# Autodesk Inventor assembly: Full Assembly
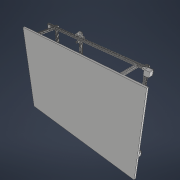
[picture p0: Inventor's stored thumbnail of the model, 180x180]
Saved by Autodesk Inventor 2022 (Build 260153000, 153)
## iProperties
Created: 2023-06-15
Part Number: Full Assembly
Document SubType Name: Assembly
Designer: Ryan Mitcham
Author: Ryan Mitcham
## Documents named in this file (21)
- C:\Users\Gaming\OneDrive\Documents\Inventor\XYZ-Gantry\Full Assembly.iam
- C:\Users\Gaming\OneDrive\Documents\Inventor\XYZ-Gantry\X-Axis.ipt
- C:\Users\Gaming\OneDrive\Documents\Inventor\XYZ-Gantry\XY-Axis Connection\XY-Axis Connection.iam
- C:\Users\Gaming\OneDrive\Documents\Inventor\XYZ-Gantry\Y-Axis.ipt
- C:\Users\Gaming\OneDrive\Documents\Inventor\XYZ-Gantry\YZ-Axis Connection\YZ-Axis Connection.iam
- C:\Users\Gaming\OneDrive\Documents\Inventor\XYZ-Gantry\Z-Axis.ipt
- C:\Users\Gaming\OneDrive\Documents\Inventor\XYZ-Gantry\Standard Parts\NEMA 17 Bi-Polar Stepper Motor.ipt
- C:\Users\Gaming\OneDrive\Documents\Inventor\XYZ-Gantry\Standard Parts\GT2 20 Teeth Motor Pulley.ipt
- C:\Users\Gaming\OneDrive\Documents\Inventor\XYZ-Gantry\Pulley Plates\X-Axis End - Straight.ipt
- C:\Users\Gaming\OneDrive\Documents\Inventor\XYZ-Gantry\Pulley Plates\Extrusion-compatible Spacer.ipt
- C:\Users\Gaming\OneDrive\Documents\Inventor\XYZ-Gantry\Standard Parts\GT2 20 Teeth Pulley.ipt
- C:\Users\Gaming\OneDrive\Documents\Inventor\XYZ-Gantry\Pulley Plates\X-Axis End - Corner.ipt
- C:\Users\Gaming\OneDrive\Documents\Inventor\XYZ-Gantry\Stepper Motor Mounting Plate.ipt
- C:\Users\Gaming\OneDrive\Documents\Inventor\XYZ-Gantry\Standard Parts\GT2 2-Side Belt Clamp.ipt
- C:\Users\Gaming\OneDrive\Documents\Inventor\XYZ-Gantry\Pulley Plates\Y-Axis Pulley Spacer.ipt
- C:\Users\Gaming\OneDrive\Documents\Inventor\XYZ-Gantry\Endstop Mounting Plate.ipt
- C:\Users\Gaming\OneDrive\Documents\Inventor\XYZ-Gantry\Support Structure\Horizontal Support.ipt
- C:\Users\Gaming\OneDrive\Documents\Inventor\XYZ-Gantry\Support Structure\Horizontal Support - Surround Bracket.ipt
- C:\Users\Gaming\OneDrive\Documents\Inventor\XYZ-Gantry\Main Carriage\Main Carriage.iam
- C:\Users\Gaming\OneDrive\Documents\Inventor\XYZ-Gantry\Support Structure\Vertical Support - with Brackets.iam
- C:\Users\Gaming\OneDrive\Documents\Inventor\XYZ-Gantry\Support Structure\Base Plate.ipt
## Components (58 placed, 20 different names)
1. X-Axis:1 — Flush:1, Flush:2, Mate:11, Mate:12, Mate:13, Mate:16, Mate:17, Flush:3, Mate:28, Flush:4, Mate:38, Flush:7, Flush:8, Flush:12, Mate:60, Mate:61, Mate:62, Mate:98, Flush:16, Mate:99, Mate:102, Flush:21, Flush:22, Mate:103, Flush:27, Mate:111, Mate:120, Flush:29, Mate:121, Flush:31
2. X-Axis:2 — Flush:1, Flush:2, Mate:14, Mate:15, Flush:5, Mate:33, Flush:6, Flush:9, Flush:10, Mate:43, Flush:11, Mate:52, Mate:53, Mate:54, Mate:79, Mate:106, Flush:23, Flush:24, Mate:108, Mate:110, Flush:26, Mate:118, Flush:28, Mate:123, Flush:32
3. XY-Axis Connection:1 [sub-assembly] — Mate:1, Mate:2, Mate:3, Mate:14, Mate:16, Mate:17
4. XY-Axis Connection:2 [sub-assembly] — Mate:4, Mate:5, Mate:6, Mate:7, Mate:15
5. Y-Axis:1 — Mate:1, Mate:2, Mate:3, Mate:4, Mate:5, Mate:6, Mate:7, Mate:18, Mate:19, Mate:77, Mate:78, Mate:96, Mate:97, Flush:18, Mate:100
6. YZ-Axis Connection:1 [sub-assembly] — Mate:18, Mate:19, Mate:22, Mate:23, Mate:24, Mate:48, Mate:49, Mate:50, Mate:73, Mate:74, Mate:75, Mate:76, Angle:1, Angle:2
7. NEMA 17 Bi-Polar Stepper Motor:1 — Mate:22, Mate:23, Mate:24, Mate:25, Mate:26
8. GT2 20 Teeth Motor Pulley:1 — Mate:25, Mate:26, Mate:51
9. X-Axis End - Straight:1 — Flush:3, Mate:28, Mate:29, Mate:30, Flush:4
10. Extrusion-compatible Spacer:1 — Mate:29, Mate:30, Mate:31, Mate:32
11. GT2 20 Teeth Pulley:1 — Mate:31, Mate:32
12. X-Axis End - Straight:2 — Flush:5, Mate:33, Flush:6, Mate:34, Mate:35
13. Extrusion-compatible Spacer:2 — Mate:34, Mate:35, Mate:36, Mate:37
14. GT2 20 Teeth Pulley:2 — Mate:36, Mate:37
15. X-Axis End - Corner:1 — Mate:38, Flush:7, Flush:8, Mate:39, Mate:40, Mate:104
16. Extrusion-compatible Spacer:3 — Mate:39, Mate:40, Mate:41, Mate:42
17. GT2 20 Teeth Pulley:3 — Mate:41, Mate:42
18. X-Axis End - Corner:2 — Flush:9, Flush:10, Mate:43, Mate:44, Mate:45, Mate:119
19. Extrusion-compatible Spacer:4 — Mate:44, Mate:45, Mate:46, Mate:47
20. GT2 20 Teeth Pulley:4 — Mate:46, Mate:47
21. Z-Axis:1 — Mate:48, Mate:49, Mate:50, Mate:51, Mate:68, Flush:13, Flush:14, Mate:101, Flush:19, Flush:20, Mate:114, Mate:115
22. Stepper Motor Mounting Plate:1 — Flush:11, Mate:52, Mate:53, Mate:54, Mate:55, Mate:56, Mate:57
23. NEMA 17 Bi-Polar Stepper Motor:2 — Mate:55, Mate:56, Mate:57, Mate:58, Mate:59
24. GT2 20 Teeth Motor Pulley:2 — Mate:58, Mate:59
25. Stepper Motor Mounting Plate:2 — Flush:12, Mate:60, Mate:61, Mate:62, Mate:63, Mate:64, Mate:65, Mate:122
26. NEMA 17 Bi-Polar Stepper Motor:3 — Mate:63, Mate:64, Mate:65, Mate:66, Mate:67
27. GT2 20 Teeth Motor Pulley:3 — Mate:66, Mate:67
28. X-Axis End - Straight:3 — Mate:68, Flush:13, Flush:14, Mate:69, Mate:70
29. Extrusion-compatible Spacer:5 — Mate:69, Mate:70, Mate:71, Mate:72
30. GT2 20 Teeth Pulley:5 — Mate:71, Mate:72
31. GT2 2-Side Belt Clamp:1 — Mate:73, Mate:74, Angle:2
32. GT2 2-Side Belt Clamp:2 — Mate:75, Mate:76, Angle:1
33. X-Axis End - Straight:4 — Mate:77, Mate:78, Mate:79, Mate:80, Mate:81, Mate:82, Mate:83
34. GT2 20 Teeth Pulley:6 — Mate:84, Mate:85
35. GT2 20 Teeth Pulley:7 — Mate:86, Mate:87
36. Y-Axis Pulley Spacer:1 — Mate:80, Mate:82, Mate:84, Mate:85
37. Y-Axis Pulley Spacer:2 — Mate:81, Mate:83, Mate:86, Mate:87
38. X-Axis End - Straight:5 — Mate:96, Mate:97, Mate:98, Flush:17
39. GT2 20 Teeth Pulley:8
40. GT2 20 Teeth Pulley:9
41. Y-Axis Pulley Spacer:3
42. Y-Axis Pulley Spacer:4
43. Endstop Mounting Plate:1 — Flush:16, Mate:99, Mate:113
44. Endstop Mounting Plate:2 — Flush:17, Flush:18, Mate:100
45. Endstop Mounting Plate:3 — Mate:101, Flush:19, Flush:20
46. Horizontal Support:1 — Mate:102, Flush:21, Mate:105, Mate:107
47. Horizontal Support - Surround Bracket:1 — Flush:22, Mate:103, Mate:104, Mate:105
48. Horizontal Support - Surround Bracket:2 — Mate:106, Flush:23, Mate:107
49. Horizontal Support:2 — Flush:24, Mate:108, Flush:25, Mate:109, Mate:112
50. Horizontal Support - Surround Bracket:3 — Flush:25, Mate:109, Mate:110, Flush:26
51. Horizontal Support - Surround Bracket:4 — Flush:27, Mate:111, Mate:112, Mate:113
52. Main Carriage:1 [sub-assembly] — Mate:114, Mate:115, Mate:116, Mate:117
53. GT2 2-Side Belt Clamp:3 — Mate:116, Mate:117
54. Vertical Support - with Brackets:1 [sub-assembly] — Mate:118, Flush:28, Mate:119, Flush:30
55. Vertical Support - with Brackets:2 [sub-assembly] — Mate:120, Flush:29, Flush:30
56. Vertical Support - with Brackets:3 [sub-assembly] — Mate:121, Flush:31, Mate:122, Flush:33
57. Vertical Support - with Brackets:4 [sub-assembly] — Mate:123, Flush:32, Flush:33, Mate:124, Flush:34, Flush:35
58. Base Plate:1 — Mate:124, Flush:34, Flush:35
## Relationships (154: Mate 118, Flush 34, Angle 2)
- Flush:1: X-Axis:1 ↔ X-Axis:2
- Flush:2: X-Axis:1 ↔ X-Axis:2
- Mate:1: XY-Axis Connection:1 ↔ Y-Axis:1
- Mate:2: XY-Axis Connection:1 ↔ Y-Axis:1
- Mate:3: XY-Axis Connection:1 ↔ Y-Axis:1
- Mate:4: XY-Axis Connection:2 ↔ Y-Axis:1
- Mate:5: XY-Axis Connection:2 ↔ Y-Axis:1
- Mate:6: XY-Axis Connection:2 ↔ Y-Axis:1
- Mate:7: XY-Axis Connection:2 ↔ Y-Axis:1
- Mate:11: X-Axis:1
- Mate:12: X-Axis:1
- Mate:13: X-Axis:1
- Mate:14 (1 mm): X-Axis:2 ↔ XY-Axis Connection:1
- Mate:15 (1 mm): X-Axis:2 ↔ XY-Axis Connection:2
- Mate:16 (1 mm): X-Axis:1 ↔ XY-Axis Connection:1
- Mate:17 (1 mm): X-Axis:1 ↔ XY-Axis Connection:1
- Mate:18 (1 mm): Y-Axis:1 ↔ YZ-Axis Connection:1
- Mate:19 (1 mm): Y-Axis:1 ↔ YZ-Axis Connection:1
- Mate:22: YZ-Axis Connection:1 ↔ NEMA 17 Bi-Polar Stepper Motor:1
- Mate:23: YZ-Axis Connection:1 ↔ NEMA 17 Bi-Polar Stepper Motor:1
- Mate:24: YZ-Axis Connection:1 ↔ NEMA 17 Bi-Polar Stepper Motor:1
- Mate:25 (10 mm): NEMA 17 Bi-Polar Stepper Motor:1 ↔ GT2 20 Teeth Motor Pulley:1
- Mate:26: NEMA 17 Bi-Polar Stepper Motor:1 ↔ GT2 20 Teeth Motor Pulley:1
- Flush:3: X-Axis:1 ↔ X-Axis End - Straight:1
- Mate:28: X-Axis:1 ↔ X-Axis End - Straight:1
- Mate:29: X-Axis End - Straight:1 ↔ Extrusion-compatible Spacer:1
- Mate:30: X-Axis End - Straight:1 ↔ Extrusion-compatible Spacer:1
- Mate:31: Extrusion-compatible Spacer:1 ↔ GT2 20 Teeth Pulley:1
- Mate:32: Extrusion-compatible Spacer:1 ↔ GT2 20 Teeth Pulley:1
- Flush:4 (20 mm): X-Axis:1 ↔ X-Axis End - Straight:1
- Flush:5: X-Axis:2 ↔ X-Axis End - Straight:2
- Mate:33: X-Axis:2 ↔ X-Axis End - Straight:2
- Flush:6 (-20 mm): X-Axis:2 ↔ X-Axis End - Straight:2
- Mate:34: X-Axis End - Straight:2 ↔ Extrusion-compatible Spacer:2
- Mate:35: X-Axis End - Straight:2 ↔ Extrusion-compatible Spacer:2
- Mate:36: Extrusion-compatible Spacer:2 ↔ GT2 20 Teeth Pulley:2
- Mate:37: Extrusion-compatible Spacer:2 ↔ GT2 20 Teeth Pulley:2
- Mate:38: X-Axis:1 ↔ X-Axis End - Corner:1
- Flush:7: X-Axis:1 ↔ X-Axis End - Corner:1
- Flush:8: X-Axis:1 ↔ X-Axis End - Corner:1
- Mate:39: X-Axis End - Corner:1 ↔ Extrusion-compatible Spacer:3
- Mate:40: X-Axis End - Corner:1 ↔ Extrusion-compatible Spacer:3
- Mate:41: Extrusion-compatible Spacer:3 ↔ GT2 20 Teeth Pulley:3
- Mate:42: Extrusion-compatible Spacer:3 ↔ GT2 20 Teeth Pulley:3
- Flush:9: X-Axis:2 ↔ X-Axis End - Corner:2
- Flush:10: X-Axis:2 ↔ X-Axis End - Corner:2
- Mate:43: X-Axis:2 ↔ X-Axis End - Corner:2
- Mate:44: X-Axis End - Corner:2 ↔ Extrusion-compatible Spacer:4
- Mate:45: X-Axis End - Corner:2 ↔ Extrusion-compatible Spacer:4
- Mate:46: Extrusion-compatible Spacer:4 ↔ GT2 20 Teeth Pulley:4
- Mate:47: Extrusion-compatible Spacer:4 ↔ GT2 20 Teeth Pulley:4
- Mate:48: YZ-Axis Connection:1 ↔ Z-Axis:1
- Mate:49 (-10 mm): YZ-Axis Connection:1 ↔ Z-Axis:1
- Mate:50 (-10 mm): YZ-Axis Connection:1 ↔ Z-Axis:1
- Mate:51 (10 mm): GT2 20 Teeth Motor Pulley:1 ↔ Z-Axis:1
- Flush:11 (-40 mm): X-Axis:2 ↔ Stepper Motor Mounting Plate:1
- Mate:52: X-Axis:2 ↔ Stepper Motor Mounting Plate:1
- Mate:53 (-10 mm): X-Axis:2 ↔ Stepper Motor Mounting Plate:1
- Mate:54 (-10 mm): X-Axis:2 ↔ Stepper Motor Mounting Plate:1
- Mate:55: Stepper Motor Mounting Plate:1 ↔ NEMA 17 Bi-Polar Stepper Motor:2
- Mate:56: Stepper Motor Mounting Plate:1 ↔ NEMA 17 Bi-Polar Stepper Motor:2
- Mate:57: Stepper Motor Mounting Plate:1 ↔ NEMA 17 Bi-Polar Stepper Motor:2
- Mate:58: NEMA 17 Bi-Polar Stepper Motor:2 ↔ GT2 20 Teeth Motor Pulley:2
- Mate:59 (2 mm): NEMA 17 Bi-Polar Stepper Motor:2 ↔ GT2 20 Teeth Motor Pulley:2
- Flush:12 (-40 mm): X-Axis:1 ↔ Stepper Motor Mounting Plate:2
- Mate:60: X-Axis:1 ↔ Stepper Motor Mounting Plate:2
- Mate:61 (-10 mm): X-Axis:1 ↔ Stepper Motor Mounting Plate:2
- Mate:62 (-10 mm): X-Axis:1 ↔ Stepper Motor Mounting Plate:2
- Mate:63: Stepper Motor Mounting Plate:2 ↔ NEMA 17 Bi-Polar Stepper Motor:3
- Mate:64: Stepper Motor Mounting Plate:2 ↔ NEMA 17 Bi-Polar Stepper Motor:3
- Mate:65: Stepper Motor Mounting Plate:2 ↔ NEMA 17 Bi-Polar Stepper Motor:3
- Mate:66: NEMA 17 Bi-Polar Stepper Motor:3 ↔ GT2 20 Teeth Motor Pulley:3
- Mate:67 (2 mm): NEMA 17 Bi-Polar Stepper Motor:3 ↔ GT2 20 Teeth Motor Pulley:3
- Mate:68: Z-Axis:1 ↔ X-Axis End - Straight:3
- Flush:13: Z-Axis:1 ↔ X-Axis End - Straight:3
- Flush:14 (-20 mm): Z-Axis:1 ↔ X-Axis End - Straight:3
- Mate:69: X-Axis End - Straight:3 ↔ Extrusion-compatible Spacer:5
- Mate:70: X-Axis End - Straight:3 ↔ Extrusion-compatible Spacer:5
- Mate:71: Extrusion-compatible Spacer:5 ↔ GT2 20 Teeth Pulley:5
- Mate:72: Extrusion-compatible Spacer:5 ↔ GT2 20 Teeth Pulley:5
- Mate:73 (1 mm): YZ-Axis Connection:1 ↔ GT2 2-Side Belt Clamp:1
- Mate:74: YZ-Axis Connection:1 ↔ GT2 2-Side Belt Clamp:1
- Mate:75: YZ-Axis Connection:1 ↔ GT2 2-Side Belt Clamp:2
- Mate:76: YZ-Axis Connection:1 ↔ GT2 2-Side Belt Clamp:2
- Mate:77: Y-Axis:1 ↔ X-Axis End - Straight:4
- Mate:78 (-10 mm): Y-Axis:1 ↔ X-Axis End - Straight:4
- Mate:79 (20 mm): X-Axis:2 ↔ X-Axis End - Straight:4
- Mate:80: X-Axis End - Straight:4 ↔ Y-Axis Pulley Spacer:1
- Mate:81: X-Axis End - Straight:4 ↔ Y-Axis Pulley Spacer:2
- Mate:82: X-Axis End - Straight:4 ↔ Y-Axis Pulley Spacer:1
- Mate:83: X-Axis End - Straight:4 ↔ Y-Axis Pulley Spacer:2
- Mate:84: GT2 20 Teeth Pulley:6 ↔ Y-Axis Pulley Spacer:1
- Mate:85: GT2 20 Teeth Pulley:6 ↔ Y-Axis Pulley Spacer:1
- Mate:86: GT2 20 Teeth Pulley:7 ↔ Y-Axis Pulley Spacer:2
- Mate:87: GT2 20 Teeth Pulley:7 ↔ Y-Axis Pulley Spacer:2
- [Mate]: X-Axis End - Straight:5 ↔ Y-Axis Pulley Spacer:3
- [Mate]: X-Axis End - Straight:5 ↔ Y-Axis Pulley Spacer:4
- [Mate]: X-Axis End - Straight:5 ↔ Y-Axis Pulley Spacer:3
- [Mate]: X-Axis End - Straight:5 ↔ Y-Axis Pulley Spacer:4
- [Mate]: GT2 20 Teeth Pulley:8 ↔ Y-Axis Pulley Spacer:3
- [Mate]: GT2 20 Teeth Pulley:8 ↔ Y-Axis Pulley Spacer:3
- [Mate]: GT2 20 Teeth Pulley:9 ↔ Y-Axis Pulley Spacer:4
- [Mate]: GT2 20 Teeth Pulley:9 ↔ Y-Axis Pulley Spacer:4
- Mate:96: Y-Axis:1 ↔ X-Axis End - Straight:5
- Mate:97 (-10 mm): Y-Axis:1 ↔ X-Axis End - Straight:5
- Mate:98 (20 mm): X-Axis:1 ↔ X-Axis End - Straight:5
- Angle:1 (90 deg): YZ-Axis Connection:1 ↔ GT2 2-Side Belt Clamp:2
- Angle:2 (90 deg): YZ-Axis Connection:1 ↔ GT2 2-Side Belt Clamp:1
- Flush:16: X-Axis:1 ↔ Endstop Mounting Plate:1
- Mate:99: X-Axis:1 ↔ Endstop Mounting Plate:1
- Flush:17 (-5 mm): X-Axis End - Straight:5 ↔ Endstop Mounting Plate:2
- Flush:18: Y-Axis:1 ↔ Endstop Mounting Plate:2
- Mate:100: Y-Axis:1 ↔ Endstop Mounting Plate:2
- Mate:101: Z-Axis:1 ↔ Endstop Mounting Plate:3
- Flush:19 (55 mm): Z-Axis:1 ↔ Endstop Mounting Plate:3
- Flush:20: Z-Axis:1 ↔ Endstop Mounting Plate:3
- Mate:102: X-Axis:1 ↔ Horizontal Support:1
- Flush:21: X-Axis:1 ↔ Horizontal Support:1
- Flush:22: X-Axis:1 ↔ Horizontal Support - Surround Bracket:1
- Mate:103: X-Axis:1 ↔ Horizontal Support - Surround Bracket:1
- Mate:104 (2 mm): X-Axis End - Corner:1 ↔ Horizontal Support - Surround Bracket:1
- Mate:105: Horizontal Support:1 ↔ Horizontal Support - Surround Bracket:1
- Mate:106: X-Axis:2 ↔ Horizontal Support - Surround Bracket:2
- Flush:23: X-Axis:2 ↔ Horizontal Support - Surround Bracket:2
- Mate:107: Horizontal Support:1 ↔ Horizontal Support - Surround Bracket:2
- Flush:24: X-Axis:2 ↔ Horizontal Support:2
- Mate:108: X-Axis:2 ↔ Horizontal Support:2
- Flush:25: Horizontal Support:2 ↔ Horizontal Support - Surround Bracket:3
- Mate:109: Horizontal Support:2 ↔ Horizontal Support - Surround Bracket:3
- Mate:110: X-Axis:2 ↔ Horizontal Support - Surround Bracket:3
- Flush:26: X-Axis:2 ↔ Horizontal Support - Surround Bracket:3
- Flush:27: X-Axis:1 ↔ Horizontal Support - Surround Bracket:4
- Mate:111: X-Axis:1 ↔ Horizontal Support - Surround Bracket:4
- Mate:112: Horizontal Support:2 ↔ Horizontal Support - Surround Bracket:4
- Mate:113: Endstop Mounting Plate:1 ↔ Horizontal Support - Surround Bracket:4
- Mate:114 (1 mm): Z-Axis:1 ↔ Main Carriage:1
- Mate:115 (1 mm): Z-Axis:1 ↔ Main Carriage:1
- Mate:116 (2 mm): Main Carriage:1 ↔ GT2 2-Side Belt Clamp:3
- Mate:117: Main Carriage:1 ↔ GT2 2-Side Belt Clamp:3
- Mate:118: X-Axis:2 ↔ Vertical Support - with Brackets:1
- Flush:28: X-Axis:2 ↔ Vertical Support - with Brackets:1
- Mate:119 (20 mm): X-Axis End - Corner:2 ↔ Vertical Support - with Brackets:1
- Mate:120: X-Axis:1 ↔ Vertical Support - with Brackets:2
- Flush:29: X-Axis:1 ↔ Vertical Support - with Brackets:2
- Flush:30: Vertical Support - with Brackets:1 ↔ Vertical Support - with Brackets:2
- Mate:121: X-Axis:1 ↔ Vertical Support - with Brackets:3
- Flush:31: X-Axis:1 ↔ Vertical Support - with Brackets:3
- Mate:122 (20 mm): Stepper Motor Mounting Plate:2 ↔ Vertical Support - with Brackets:3
- Mate:123: X-Axis:2 ↔ Vertical Support - with Brackets:4
- Flush:32: X-Axis:2 ↔ Vertical Support - with Brackets:4
- Flush:33: Vertical Support - with Brackets:3 ↔ Vertical Support - with Brackets:4
- Mate:124: Vertical Support - with Brackets:4 ↔ Base Plate:1
- Flush:34 (10 mm): Vertical Support - with Brackets:4 ↔ Base Plate:1
- Flush:35 (200 mm): Vertical Support - with Brackets:4 ↔ Base Plate:1
## Named parameters: d116_d108 = 0 mm, d117_d109 = 0 mm, d118_d110 = 0 mm, d119_d111 = 0 mm, d120_d112 = 0 mm, d121_d113 = 0 mm, d122_d114 = 0 mm, d123_d115 = 0 mm
